# Autodesk Inventor assembly: 20-J2
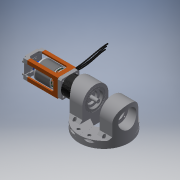
[picture p0: Inventor's stored thumbnail of the model, 180x180]
Saved by Autodesk Inventor 2018 (Build 220112000, 112)
## iProperties
Created: 2020-01-14
Part Number: 20-J2
Document SubType Name: Assembly
Designer: Bunny320
Author: Bunny320
## Documents named in this file (5)
- C:\Users\Bunny320\Desktop\sechs\4-CAD\20-J2.iam
- C:\Users\Bunny320\Desktop\sechs\4-CAD\201-flange-with motor.ipt
- C:\Users\Bunny320\Desktop\sechs\4-CAD\standardParts\61807-2RS1\61807-2RS1.iam
- C:\Users\Bunny320\Desktop\sechs\4-CAD\motor unit.iam
- C:\Users\Bunny320\Desktop\sechs\4-CAD\202-flange adapter.ipt
## Components (6 placed, 4 different names)
1. 201-flange-with motor:1 — Flush:1, Flush:2, Flush:3, Mate:1, Mate:2, Flush:4, Mate:3, Mate:4, Mate:7, Mate:8, Mate:9, Mate:10, Mate:11, Mate:12
2. 201-flange-with motor:2 — Mate:1, Mate:2, Flush:4, Mate:5, Mate:6
3. 61807-2RS1:1 [sub-assembly] — Mate:3, Mate:4
4. 61807-2RS1:2 [sub-assembly] — Mate:5, Mate:6
5. motor unit:1 [sub-assembly] — Mate:7, Mate:8, Mate:9
6. 202-flange adapter:1 — Mate:10, Mate:11, Mate:12
## Relationships (16: Mate 12, Flush 4)
- Flush:1: 201-flange-with motor:1
- Flush:2: 201-flange-with motor:1
- Flush:3: 201-flange-with motor:1
- Mate:1: 201-flange-with motor:1 ↔ 201-flange-with motor:2
- Mate:2: 201-flange-with motor:1 ↔ 201-flange-with motor:2
- Flush:4: 201-flange-with motor:1 ↔ 201-flange-with motor:2
- Mate:3: 201-flange-with motor:1 ↔ 61807-2RS1:1
- Mate:4: 201-flange-with motor:1 ↔ 61807-2RS1:1
- Mate:5: 201-flange-with motor:2 ↔ 61807-2RS1:2
- Mate:6: 201-flange-with motor:2 ↔ 61807-2RS1:2
- Mate:7: 201-flange-with motor:1 ↔ motor unit:1
- Mate:8: 201-flange-with motor:1 ↔ motor unit:1
- Mate:9: 201-flange-with motor:1 ↔ motor unit:1
- Mate:10: 201-flange-with motor:1 ↔ 202-flange adapter:1
- Mate:11: 201-flange-with motor:1 ↔ 202-flange adapter:1
- Mate:12: 201-flange-with motor:1 ↔ 202-flange adapter:1
